# Autodesk Inventor assembly: Humanóide - rev0
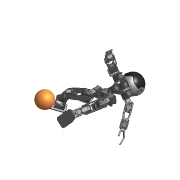
[picture p0: Inventor's stored thumbnail of the model, 180x180]
Saved by Autodesk Inventor 2011 (Build 150239000, 239)
## iProperties
Created: 2010-11-21
Part Number: Humanóide - rev0
Document SubType Name: Assembly
Designer: Milton
Mass: 1911.62 g
Surface Area: 4804 cm^2
Volume: 1270.78 cm^3
Density: 1.50429 g/cm^3
Author: Milton
## Documents named in this file (30)
- C:\Users\Milton\Documents\Futbots\IC - Humanóide\Desenhos\Humanóide - rev0.iam
- C:\Users\Milton\Documents\Futbots\IC - Humanóide\Desenhos\Right foot.ipt
- C:\Users\Milton\Documents\Futbots\IC - Humanóide\Desenhos\Imported Components\RX-28\RX-28.ipt
- C:\Users\Milton\Documents\Futbots\IC - Humanóide\Desenhos\Imported Components\RX-28 Horn\RX-28 Horn.ipt
- C:\Users\Milton\Documents\Futbots\IC - Humanóide\Desenhos\Ankle.ipt
- C:\Users\Milton\Documents\Futbots\IC - Humanóide\Desenhos\Hips.ipt
- C:\Users\Milton\Documents\Futbots\IC - Humanóide\Desenhos\Thigh.ipt
- C:\Users\Milton\Documents\Futbots\IC - Humanóide\Desenhos\Left foot.ipt
- C:\Users\Milton\Documents\Futbots\IC - Humanóide\Desenhos\Knee - Back.ipt
- C:\Users\Milton\Documents\Futbots\IC - Humanóide\Desenhos\Knee - Front.ipt
- C:\Users\Milton\Documents\Futbots\IC - Humanóide\Desenhos\Groin.ipt
- C:\Users\Milton\Documents\Futbots\IC - Humanóide\Desenhos\Pelvis.ipt
- C:\Users\Milton\Documents\Futbots\IC - Humanóide\Desenhos\Waistline.ipt
- C:\Users\Milton\Documents\Futbots\IC - Humanóide\Desenhos\Trunk.ipt
- C:\Users\Milton\Documents\Futbots\IC - Humanóide\Desenhos\Shoulder.ipt
- C:\Users\Milton\Documents\Futbots\IC - Humanóide\Desenhos\Arm.ipt
- C:\Users\Milton\Documents\Futbots\IC - Humanóide\Desenhos\Trapezium.ipt
- C:\Users\Milton\Documents\Futbots\IC - Humanóide\Desenhos\Right Hand.ipt
- C:\Users\Milton\Documents\Futbots\IC - Humanóide\Desenhos\Left Hand.ipt
- C:\Users\Milton\Documents\Futbots\IC - Humanóide\Desenhos\Alça.ipt
- C:\Users\Milton\Documents\Futbots\IC - Humanóide\Desenhos\Neck.ipt
- C:\Users\Milton\Documents\Inventor\Content Center Files\R2011\en-US\ISO 7380\ISO 7380 - M3 x 6.ipt
- C:\Users\Milton\Documents\Futbots\IC - Humanóide\Desenhos\Head.iam
- C:\Users\Milton\Documents\Futbots\IC - Humanóide\Desenhos\Ball.ipt
- C:\Users\Milton\Documents\Futbots\IC - Humanóide\Desenhos\Humanóide - rev0\AIP\Stress Analysis\{6B0C443B-3575-4766-89EC-E2AB749BE7BF}\Brep_0\Humanóide - rev0_INS_{7D960F55-6937-454E-B973-146CFB6E3506}.fins
- C:\Users\Milton\Documents\Futbots\IC - Humanóide\Desenhos\Humanóide - rev0\AIP\Stress Analysis\{6B0C443B-3575-4766-89EC-E2AB749BE7BF}\Brep_0\Humanóide - rev0_sat_{44389967-61AA-4BE1-B7EC-D3EA2D2FE9C6}.fsat
- C:\Users\Milton\Documents\Futbots\IC - Humanóide\Desenhos\Humanóide - rev0\AIP\Stress Analysis\{6B0C443B-3575-4766-89EC-E2AB749BE7BF}\Brep_0\Humanóide - rev0_tes_{B0B6FCF0-E664-439E-BE88-AB80D02FF4B7}.ftes
- C:\Users\Milton\Documents\Futbots\IC - Humanóide\Desenhos\Humanóide - rev0\AIP\Stress Analysis\{6B0C443B-3575-4766-89EC-E2AB749BE7BF}\Brep_0\Humanóide - rev0_wiz_{24C38105-2EA3-4ABB-8DFC-E581D1C3461D}.fwiz
- C:\Users\Milton\Documents\Futbots\IC - Humanóide\Desenhos\Humanóide - rev0\AIP\Stress Analysis\{6B0C443B-3575-4766-89EC-E2AB749BE7BF}\Simulation_0\Humanóide - rev0_msh_{642BD46C-0DBD-4A00-9AC0-F0BB7B45041F}.fmsh
- C:\Users\Milton\Documents\Futbots\IC - Humanóide\Desenhos\Humanóide - rev0\AIP\Stress Analysis\{6B0C443B-3575-4766-89EC-E2AB749BE7BF}\Simulation_0\Humanóide - rev0_res_{B27E6E0C-00E3-4C61-99AA-CF472A861E25}.fres
## Components (147 placed, 23 different names)
1. RX-28:1 — Mate:58, Mate:59, Mate:60, Mate:67, Mate:68, Mate:73
2. RX-28:2 — Mate:55, Mate:56, Mate:57, Mate:69, Mate:70, Mate:76
3. RX-28:3 — Mate:80, Mate:81, Mate:82, Mate:83, Mate:84, Mate:85, Mate:86, Mate:87, Flush:7, Mate:128, Mate:211
4. RX-28:4 — Mate:88, Mate:89, Mate:90, Mate:97, Mate:98, Flush:9, Mate:129, Mate:130, Flush:13, Insert:22, Insert:23
5. RX-28:5 — Mate:91, Mate:92, Mate:93, Mate:95, Mate:96, Mate:131, Mate:200, Mate:201, Insert:37, Insert:38, Insert:62
6. RX-28:6 — Flush:7, Mate:128, Flush:9, Mate:132, Mate:133, Mate:196, Mate:197
7. RX-28 Horn:1 — Mate:4, Mate:5, Mate:159, Mate:160, Mate:161
8. RX-28 Horn:2 — Mate:6, Mate:7, Mate:180, Mate:181, Mate:182, Mate:194, Mate:195
9. RX-28 Horn:3 — Mate:8, Mate:10, Mate:12, Mate:14, Flush:3, Flush:4, Mate:31
10. RX-28 Horn:4 — Mate:16, Mate:19, Mate:20, Flush:5, Flush:6, Mate:34
11. RX-28 Horn:5 — Mate:15, Mate:17, Mate:18, Mate:21, Mate:177, Mate:178, Mate:179, Mate:191, Mate:192, Mate:193, Insert:9, Insert:10, Insert:48, Insert:49, Insert:85, Insert:86
12. RX-28 Horn:6 — Mate:32, Flush:5, Flush:6, Mate:127
13. RX-28 Horn:7 — Mate:99, Mate:100, Flush:10, Mate:168, Mate:169, Mate:170, Mate:171, Mate:172
14. RX-28 Horn:8 — Mate:27, Mate:28, Mate:175, Mate:184, Mate:185, Mate:189, Mate:190
15. RX-28 Horn:9 — Mate:101, Mate:102, Mate:144, Mate:145, Mate:147, Mate:148, Mate:164, Mate:165
16. RX-28 Horn:10 — Mate:9, Mate:11, Mate:13, Mate:173, Mate:174, Mate:183, Mate:186, Mate:187, Mate:188, Insert:11, Insert:12, Insert:46, Insert:47, Insert:77, Insert:79, Insert:83, Insert:84
17. RX-28 Horn:11 — Flush:10, Mate:141, Mate:153, Mate:154, Mate:155, Mate:166, Mate:167, Insert:42, Insert:43, Insert:91, Insert:92
18. RX-28 Horn:16 — Mate:61, Mate:62, Mate:63, Mate:64, Mate:65, Mate:66, Mate:72, Mate:74, Mate:75, Mate:77, Mate:78, Mate:79, Mate:212
19. RX-28 Horn:17 — Mate:29, Flush:3, Flush:4, Mate:126
20. RX-28 Horn:19 — Mate:149, Mate:150, Mate:156, Mate:157, Mate:208, Insert:87, Insert:88, Insert:89, Insert:90
21. RX-28 Horn:21 — Mate:22, Mate:25, Mate:26, Mate:162, Mate:163
22. RX-28 Horn:22 — Mate:198, Mate:199, Mate:213
23. Ankle:1 — Mate:4, Mate:5, Mate:6, Mate:7
24. Ankle:2 — Mate:25, Mate:26, Mate:27, Mate:28
25. Hips:1 — Mate:32, Mate:34, Mate:69, Mate:70, Mate:127
26. Hips:2 — Mate:29, Mate:31, Mate:67, Mate:68, Mate:126
27. Thigh:1 — Mate:8, Mate:9, Mate:10, Mate:11
28. Thigh:2 — Mate:12, Mate:13, Mate:14
29. Thigh:3 — Mate:15, Mate:16, Mate:17
30. Thigh:4 — Mate:18, Mate:19, Mate:20, Mate:21
31. Waistline:1 — Mate:78, Mate:79, Mate:80, Mate:81
32. Right foot:1 — Mate:159, Mate:160, Mate:161, Insert:16, Insert:17, Insert:68, Insert:69, Mate:210
33. Left foot:1 — Mate:22, Mate:162, Mate:163, Mate:202, Mate:203, Insert:15, Insert:70, Insert:71, Insert:72, Mate:209
34. Knee - Back:1 — Mate:186, Mate:187, Mate:188, Mate:189, Mate:190, Insert:18, Insert:19
35. Knee - Front:1 — Mate:173, Mate:174, Mate:175, Mate:183, Mate:184, Mate:185, Insert:75, Insert:76
36. Knee - Front:2 — Mate:177, Mate:178, Mate:179, Mate:180, Mate:181, Mate:182, Insert:73, Insert:74
37. Groin:1 — Mate:55, Mate:56, Mate:57, Mate:64, Mate:65, Mate:66, Insert:32, Insert:36, Insert:52, Insert:53
38. Groin:2 — Mate:58, Mate:59, Mate:60, Mate:61, Mate:62, Mate:63, Insert:44, Insert:45, Insert:50, Insert:51
39. Pelvis:1 — Mate:75, Mate:76, Mate:77, Insert:30, Insert:31, Insert:34, Insert:35
40. Pelvis:2 — Mate:72, Mate:73, Mate:74, Insert:13, Insert:14, Insert:33, Mate:204, Mate:205
41. Trunk:1 — Mate:82, Mate:83, Mate:84, Mate:88, Mate:89, Mate:90, Insert:28, Insert:29, Insert:54, Insert:55
42. Trunk:2 — Mate:85, Mate:86, Mate:87, Mate:91, Mate:92, Mate:93, Insert:24, Insert:25, Insert:26, Insert:27
43. Shoulder:1 — Mate:97, Mate:98, Mate:101, Mate:102
44. Shoulder:2 — Mate:95, Mate:96, Mate:99, Mate:100
45. Trapezium:1 — Mate:129, Mate:130, Insert:56, Insert:57, Insert:58, Insert:63
46. Trapezium:2 — Mate:131, Mate:132, Mate:133, Insert:59, Insert:60
47. Right Hand:1 — Mate:153, Mate:154, Mate:155
48. Arm:3 — Mate:170, Mate:171, Mate:172, Insert:39, Insert:40, Mate:206, Mate:207, Insert:41
49. Arm:4 — Mate:147, Mate:148, Mate:165, Insert:5, Insert:6, Insert:7, Insert:8
50. Arm:6 — Mate:141, Mate:166, Mate:167, Mate:168, Mate:169, Insert:64, Insert:65, Insert:66, Insert:67
51. Arm:7 — Mate:144, Mate:145, Mate:149, Mate:150, Mate:164, Insert:1, Insert:2, Insert:3, Insert:4
52. Left Hand:1 — Mate:156, Mate:157, Mate:208
53. Knee - Back:2 — Mate:191, Mate:192, Mate:193, Mate:194, Mate:195, Insert:20, Insert:21
54. Alça:1 — Flush:13, Mate:200, Mate:201
55. Neck:1 — Mate:196, Mate:197, Mate:198, Mate:199, Flush:14
56. Head:1 [sub-assembly] — Mate:213, Flush:14
57. Ball:1
58. ISO 7380 M3 x 6:1 — Insert:1
59. ISO 7380 M3 x 6:2 — Insert:2
60. ISO 7380 M3 x 6:3 — Insert:3
61. ISO 7380 M3 x 6:4 — Insert:4
62. ISO 7380 M3 x 6:5 — Insert:5
63. ISO 7380 M3 x 6:6 — Insert:6
64. ISO 7380 M3 x 6:7 — Insert:7
65. ISO 7380 M3 x 6:8 — Insert:8
66. ISO 7380 M3 x 6:9 — Insert:9
67. ISO 7380 M3 x 6:10 — Insert:10
68. ISO 7380 M3 x 6:11 — Insert:11
69. ISO 7380 M3 x 6:12 — Insert:12
70. ISO 7380 M3 x 6:13 — Insert:13
71. ISO 7380 M3 x 6:14 — Insert:14
72. ISO 7380 M3 x 6:15 — Mate:202, Mate:203
73. ISO 7380 M3 x 6:16 — Insert:15
74. ISO 7380 M3 x 6:17 — Insert:16
75. ISO 7380 M3 x 6:18 — Insert:17
76. ISO 7380 M3 x 6:19 — Insert:18
77. ISO 7380 M3 x 6:20 — Insert:19
78. ISO 7380 M3 x 6:21 — Insert:20
79. ISO 7380 M3 x 6:22 — Insert:21
80. ISO 7380 M3 x 6:23 — Insert:22
81. ISO 7380 M3 x 6:24 — Insert:23
82. ISO 7380 M3 x 6:25 — Insert:24
83. ISO 7380 M3 x 6:26 — Insert:25
84. ISO 7380 M3 x 6:27 — Insert:26
85. ISO 7380 M3 x 6:28 — Insert:27
86. ISO 7380 M3 x 6:29 — Insert:28
87. ISO 7380 M3 x 6:30 — Insert:29
88. ISO 7380 M3 x 6:31 — Insert:30
89. ISO 7380 M3 x 6:32 — Insert:31
90. ISO 7380 M3 x 6:33 — Insert:32
91. ISO 7380 M3 x 6:34 — Insert:33
92. ISO 7380 M3 x 6:35 — Mate:204, Mate:205
93. ISO 7380 M3 x 6:36 — Insert:34
94. ISO 7380 M3 x 6:37 — Insert:35
95. ISO 7380 M3 x 6:38 — Insert:36
96. ISO 7380 M3 x 6:39 — Insert:37
97. ISO 7380 M3 x 6:40 — Insert:38
98. ISO 7380 M3 x 6:41 — Insert:39
99. ISO 7380 M3 x 6:42 — Insert:40
100. ISO 7380 M3 x 6:43 — Mate:206, Mate:207
101. ISO 7380 M3 x 6:44 — Insert:41
102. ISO 7380 M3 x 6:45 — Insert:42
103. ISO 7380 M3 x 6:46 — Insert:43
104. ISO 7380 M3 x 6:47 — Insert:44
105. ISO 7380 M3 x 6:48 — Insert:45
106. ISO 7380 M3 x 6:49 — Insert:46
107. ISO 7380 M3 x 6:50 — Insert:47
108. ISO 7380 M3 x 6:51 — Insert:48
109. ISO 7380 M3 x 6:52 — Insert:49
110. ISO 7380 M3 x 6:53 — Insert:50
111. ISO 7380 M3 x 6:54 — Insert:51
112. ISO 7380 M3 x 6:55 — Insert:52
113. ISO 7380 M3 x 6:56 — Insert:53
114. ISO 7380 M3 x 6:57 — Insert:54
115. ISO 7380 M3 x 6:58 — Insert:55
116. ISO 7380 M3 x 6:59 — Insert:56
117. ISO 7380 M3 x 6:60 — Insert:57
118. ISO 7380 M3 x 6:61 — Insert:58
119. ISO 7380 M3 x 6:62 — Insert:59
120. ISO 7380 M3 x 6:63 — Insert:60
121. ISO 7380 M3 x 6:65 — Insert:62
122. ISO 7380 M3 x 6:66 — Insert:63
123. ISO 7380 M3 x 6:67 — Insert:64
124. ISO 7380 M3 x 6:68 — Insert:65
125. ISO 7380 M3 x 6:69 — Insert:66
126. ISO 7380 M3 x 6:70 — Insert:67
127. ISO 7380 M3 x 6:71 — Insert:68
128. ISO 7380 M3 x 6:72 — Insert:69
129. ISO 7380 M3 x 6:73 — Insert:70
130. ISO 7380 M3 x 6:74 — Insert:71
131. ISO 7380 M3 x 6:75 — Insert:72
132. ISO 7380 M3 x 6:76 — Insert:73
133. ISO 7380 M3 x 6:77 — Insert:74
134. ISO 7380 M3 x 6:78 — Insert:75
135. ISO 7380 M3 x 6:79 — Insert:76
136. ISO 7380 M3 x 6:80 — Insert:77
137. ISO 7380 M3 x 6:82 — Insert:79
138. ISO 7380 M3 x 6:86 — Insert:83
139. ISO 7380 M3 x 6:87 — Insert:84
140. ISO 7380 M3 x 6:88 — Insert:85
141. ISO 7380 M3 x 6:89 — Insert:86
142. ISO 7380 M3 x 6:90 — Insert:87
143. ISO 7380 M3 x 6:91 — Insert:88
144. ISO 7380 M3 x 6:92 — Insert:89
145. ISO 7380 M3 x 6:93 — Insert:90
146. ISO 7380 M3 x 6:94 — Insert:91
147. ISO 7380 M3 x 6:95 — Insert:92
## Relationships (243: Mate 147, Insert 87, Flush 9)
- Mate:4: RX-28 Horn:1 ↔ Ankle:1
- Mate:5: RX-28 Horn:1 ↔ Ankle:1
- Mate:6: RX-28 Horn:2 ↔ Ankle:1
- Mate:7: RX-28 Horn:2 ↔ Ankle:1
- Mate:8: RX-28 Horn:3 ↔ Thigh:1
- Mate:9: RX-28 Horn:10 ↔ Thigh:1
- Mate:10: RX-28 Horn:3 ↔ Thigh:1
- Mate:11: RX-28 Horn:10 ↔ Thigh:1
- Mate:12: RX-28 Horn:3 ↔ Thigh:2
- Mate:13: RX-28 Horn:10 ↔ Thigh:2
- Mate:14: RX-28 Horn:3 ↔ Thigh:2
- Mate:15: RX-28 Horn:5 ↔ Thigh:3
- Mate:16: RX-28 Horn:4 ↔ Thigh:3
- Mate:17: RX-28 Horn:5 ↔ Thigh:3
- Mate:18: RX-28 Horn:5 ↔ Thigh:4
- Mate:19: RX-28 Horn:4 ↔ Thigh:4
- Mate:20: RX-28 Horn:4 ↔ Thigh:4
- Mate:21: RX-28 Horn:5 ↔ Thigh:4
- Mate:22: RX-28 Horn:21 ↔ Left foot:1
- Mate:25: RX-28 Horn:21 ↔ Ankle:2
- Mate:26: RX-28 Horn:21 ↔ Ankle:2
- Mate:27: RX-28 Horn:8 ↔ Ankle:2
- Mate:28: RX-28 Horn:8 ↔ Ankle:2
- Mate:29: RX-28 Horn:17 ↔ Hips:2
- Flush:3: RX-28 Horn:3 ↔ RX-28 Horn:17
- Flush:4: RX-28 Horn:3 ↔ RX-28 Horn:17
- Mate:31 (3 mm): RX-28 Horn:3 ↔ Hips:2
- Mate:32: RX-28 Horn:6 ↔ Hips:1
- Flush:5: RX-28 Horn:4 ↔ RX-28 Horn:6
- Flush:6: RX-28 Horn:4 ↔ RX-28 Horn:6
- Mate:34 (3 mm): RX-28 Horn:4 ↔ Hips:1
- Mate:55: RX-28:2 ↔ Groin:1
- Mate:56: RX-28:2 ↔ Groin:1
- Mate:57: RX-28:2 ↔ Groin:1
- Mate:58: RX-28:1 ↔ Groin:2
- Mate:59: RX-28:1 ↔ Groin:2
- Mate:60: RX-28:1 ↔ Groin:2
- Mate:61: RX-28 Horn:16 ↔ Groin:2
- Mate:62: RX-28 Horn:16 ↔ Groin:2
- Mate:63: RX-28 Horn:16 ↔ Groin:2
- Mate:64: RX-28 Horn:16 ↔ Groin:1
- Mate:65: RX-28 Horn:16 ↔ Groin:1
- Mate:66: RX-28 Horn:16 ↔ Groin:1
- Mate:67: RX-28:1 ↔ Hips:2
- Mate:68: RX-28:1 ↔ Hips:2
- Mate:69: RX-28:2 ↔ Hips:1
- Mate:70: RX-28:2 ↔ Hips:1
- Mate:72: RX-28 Horn:16 ↔ Pelvis:2
- Mate:73: RX-28:1 ↔ Pelvis:2
- Mate:74: RX-28 Horn:16 ↔ Pelvis:2
- Mate:75: RX-28 Horn:16 ↔ Pelvis:1
- Mate:76: RX-28:2 ↔ Pelvis:1
- Mate:77: RX-28 Horn:16 ↔ Pelvis:1
- Mate:78: RX-28 Horn:16 ↔ Waistline:1
- Mate:79: RX-28 Horn:16 ↔ Waistline:1
- Mate:80: RX-28:3 ↔ Waistline:1
- Mate:81: RX-28:3 ↔ Waistline:1
- Mate:82: RX-28:3 ↔ Trunk:1
- Mate:83: RX-28:3 ↔ Trunk:1
- Mate:84: RX-28:3 ↔ Trunk:1
- Mate:85: RX-28:3 ↔ Trunk:2
- Mate:86: RX-28:3 ↔ Trunk:2
- Mate:87: RX-28:3 ↔ Trunk:2
- Mate:88: RX-28:4 ↔ Trunk:1
- Mate:89: RX-28:4 ↔ Trunk:1
- Mate:90: RX-28:4 ↔ Trunk:1
- Mate:91: RX-28:5 ↔ Trunk:2
- Mate:92: RX-28:5 ↔ Trunk:2
- Mate:93: RX-28:5 ↔ Trunk:2
- Mate:95: RX-28:5 ↔ Shoulder:2
- Mate:96: RX-28:5 ↔ Shoulder:2
- Mate:97: RX-28:4 ↔ Shoulder:1
- Mate:98: RX-28:4 ↔ Shoulder:1
- Mate:99: RX-28 Horn:7 ↔ Shoulder:2
- Mate:100: RX-28 Horn:7 ↔ Shoulder:2
- Mate:101: RX-28 Horn:9 ↔ Shoulder:1
- Mate:102: RX-28 Horn:9 ↔ Shoulder:1
- Mate:126: RX-28 Horn:17 ↔ Hips:2
- Mate:127: RX-28 Horn:6 ↔ Hips:1
- Flush:7: RX-28:3 ↔ RX-28:6
- Mate:128: RX-28:3 ↔ RX-28:6
- Flush:9: RX-28:4 ↔ RX-28:6
- Mate:129: RX-28:4 ↔ Trapezium:1
- Mate:130: RX-28:4 ↔ Trapezium:1
- Mate:131: RX-28:5 ↔ Trapezium:2
- Mate:132: RX-28:6 ↔ Trapezium:2
- Mate:133: RX-28:6 ↔ Trapezium:2
- Flush:10: RX-28 Horn:7 ↔ RX-28 Horn:11
- Mate:141: RX-28 Horn:11 ↔ Arm:6
- Mate:144: RX-28 Horn:9 ↔ Arm:7
- Mate:145: RX-28 Horn:9 ↔ Arm:7
- Mate:147: RX-28 Horn:9 ↔ Arm:4
- Mate:148: RX-28 Horn:9 ↔ Arm:4
- Mate:149: RX-28 Horn:19 ↔ Arm:7
- Mate:150: RX-28 Horn:19 ↔ Arm:7
- Mate:153: RX-28 Horn:11 ↔ Right Hand:1
- Mate:154: RX-28 Horn:11 ↔ Right Hand:1
- Mate:155: RX-28 Horn:11 ↔ Right Hand:1
- Mate:156: RX-28 Horn:19 ↔ Left Hand:1
- Mate:157: RX-28 Horn:19 ↔ Left Hand:1
- Mate:159: RX-28 Horn:1 ↔ Right foot:1
- Mate:160: RX-28 Horn:1 ↔ Right foot:1
- Mate:161: RX-28 Horn:1 ↔ Right foot:1
- Mate:162: RX-28 Horn:21 ↔ Left foot:1
- Mate:163: RX-28 Horn:21 ↔ Left foot:1
- Mate:164: RX-28 Horn:9 ↔ Arm:7
- Mate:165: RX-28 Horn:9 ↔ Arm:4
- Mate:166: RX-28 Horn:11 ↔ Arm:6
- Mate:167: RX-28 Horn:11 ↔ Arm:6
- Mate:168: RX-28 Horn:7 ↔ Arm:6
- Mate:169: RX-28 Horn:7 ↔ Arm:6
- Mate:170: RX-28 Horn:7 ↔ Arm:3
- Mate:171: RX-28 Horn:7 ↔ Arm:3
- Mate:172: RX-28 Horn:7 ↔ Arm:3
- Mate:173: RX-28 Horn:10 ↔ Knee - Front:1
- Mate:174: RX-28 Horn:10 ↔ Knee - Front:1
- Mate:175: RX-28 Horn:8 ↔ Knee - Front:1
- Mate:177: RX-28 Horn:5 ↔ Knee - Front:2
- Mate:178: RX-28 Horn:5 ↔ Knee - Front:2
- Mate:179: RX-28 Horn:5 ↔ Knee - Front:2
- Mate:180: RX-28 Horn:2 ↔ Knee - Front:2
- Mate:181: RX-28 Horn:2 ↔ Knee - Front:2
- Mate:182: RX-28 Horn:2 ↔ Knee - Front:2
- Mate:183: RX-28 Horn:10 ↔ Knee - Front:1
- Mate:184: RX-28 Horn:8 ↔ Knee - Front:1
- Mate:185: RX-28 Horn:8 ↔ Knee - Front:1
- Mate:186: RX-28 Horn:10 ↔ Knee - Back:1
- Mate:187: RX-28 Horn:10 ↔ Knee - Back:1
- Mate:188: RX-28 Horn:10 ↔ Knee - Back:1
- Mate:189: RX-28 Horn:8 ↔ Knee - Back:1
- Mate:190: RX-28 Horn:8 ↔ Knee - Back:1
- Mate:191: RX-28 Horn:5 ↔ Knee - Back:2
- Mate:192: RX-28 Horn:5 ↔ Knee - Back:2
- Mate:193: RX-28 Horn:5 ↔ Knee - Back:2
- Mate:194: RX-28 Horn:2 ↔ Knee - Back:2
- Mate:195: RX-28 Horn:2 ↔ Knee - Back:2
- Flush:13: RX-28:4 ↔ Alça:1
- Mate:196: RX-28:6 ↔ Neck:1
- Mate:197: RX-28:6 ↔ Neck:1
- Mate:198: RX-28 Horn:22 ↔ Neck:1
- Mate:199: RX-28 Horn:22 ↔ Neck:1
- Mate:200: RX-28:5 ↔ Alça:1
- Mate:201: RX-28:5 ↔ Alça:1
- Mate:203: Left foot:1 ↔ ISO 7380 M3 x 6:15
- Mate:205: Pelvis:2 ↔ ISO 7380 M3 x 6:35
- Mate:207: Arm:3 ↔ ISO 7380 M3 x 6:43
- Mate:208: RX-28 Horn:19 ↔ Left Hand:1
- Mate:209: Left foot:1
- Mate:210: Right foot:1
- Mate:211: RX-28:3
- Mate:212 (-15 mm): RX-28 Horn:16
- Mate:213: RX-28 Horn:22 ↔ Head:1
- Flush:14 (-35.5 mm): Neck:1 ↔ Head:1
- Insert:1: Arm:7 ↔ ISO 7380 M3 x 6:1
- Insert:2: Arm:7 ↔ ISO 7380 M3 x 6:2
- Insert:3: Arm:7 ↔ ISO 7380 M3 x 6:3
- Insert:4: Arm:7 ↔ ISO 7380 M3 x 6:4
- Insert:5: Arm:4 ↔ ISO 7380 M3 x 6:5
- Insert:6: Arm:4 ↔ ISO 7380 M3 x 6:6
- Insert:7: Arm:4 ↔ ISO 7380 M3 x 6:7
- Insert:8: Arm:4 ↔ ISO 7380 M3 x 6:8
- Insert:9: RX-28 Horn:5 ↔ ISO 7380 M3 x 6:9
- Insert:10: RX-28 Horn:5 ↔ ISO 7380 M3 x 6:10
- Insert:11: RX-28 Horn:10 ↔ ISO 7380 M3 x 6:11
- Insert:12: RX-28 Horn:10 ↔ ISO 7380 M3 x 6:12
- Insert:13: Pelvis:2 ↔ ISO 7380 M3 x 6:13
- Insert:14: Pelvis:2 ↔ ISO 7380 M3 x 6:14
- Mate:202: Left foot:1 ↔ ISO 7380 M3 x 6:15
- Insert:15: Left foot:1 ↔ ISO 7380 M3 x 6:16
- Insert:16: Right foot:1 ↔ ISO 7380 M3 x 6:17
- Insert:17: Right foot:1 ↔ ISO 7380 M3 x 6:18
- Insert:18: Knee - Back:1 ↔ ISO 7380 M3 x 6:19
- Insert:19: Knee - Back:1 ↔ ISO 7380 M3 x 6:20
- Insert:20: Knee - Back:2 ↔ ISO 7380 M3 x 6:21
- Insert:21: Knee - Back:2 ↔ ISO 7380 M3 x 6:22
- Insert:22: RX-28:4 ↔ ISO 7380 M3 x 6:23
- Insert:23: RX-28:4 ↔ ISO 7380 M3 x 6:24
- Insert:24: Trunk:2 ↔ ISO 7380 M3 x 6:25
- Insert:25: Trunk:2 ↔ ISO 7380 M3 x 6:26
- Insert:26: Trunk:2 ↔ ISO 7380 M3 x 6:27
- Insert:27: Trunk:2 ↔ ISO 7380 M3 x 6:28
- Insert:28: Trunk:1 ↔ ISO 7380 M3 x 6:29
- Insert:29: Trunk:1 ↔ ISO 7380 M3 x 6:30
- Insert:30: Pelvis:1 ↔ ISO 7380 M3 x 6:31
- Insert:31: Pelvis:1 ↔ ISO 7380 M3 x 6:32
- Insert:32: Groin:1 ↔ ISO 7380 M3 x 6:33
- Insert:33: Pelvis:2 ↔ ISO 7380 M3 x 6:34
- Mate:204: Pelvis:2 ↔ ISO 7380 M3 x 6:35
- Insert:34: Pelvis:1 ↔ ISO 7380 M3 x 6:36
- Insert:35: Pelvis:1 ↔ ISO 7380 M3 x 6:37
- Insert:36: Groin:1 ↔ ISO 7380 M3 x 6:38
- Insert:37: RX-28:5 ↔ ISO 7380 M3 x 6:39
- Insert:38: RX-28:5 ↔ ISO 7380 M3 x 6:40
- Insert:39: Arm:3 ↔ ISO 7380 M3 x 6:41
- Insert:40: Arm:3 ↔ ISO 7380 M3 x 6:42
- Mate:206: Arm:3 ↔ ISO 7380 M3 x 6:43
- Insert:41: Arm:3 ↔ ISO 7380 M3 x 6:44
- Insert:42: RX-28 Horn:11 ↔ ISO 7380 M3 x 6:45
- Insert:43: RX-28 Horn:11 ↔ ISO 7380 M3 x 6:46
- Insert:44: Groin:2 ↔ ISO 7380 M3 x 6:47
- Insert:45: Groin:2 ↔ ISO 7380 M3 x 6:48
- Insert:46: RX-28 Horn:10 ↔ ISO 7380 M3 x 6:49
- Insert:47: RX-28 Horn:10 ↔ ISO 7380 M3 x 6:50
- Insert:48: RX-28 Horn:5 ↔ ISO 7380 M3 x 6:51
- Insert:49: RX-28 Horn:5 ↔ ISO 7380 M3 x 6:52
- Insert:50: Groin:2 ↔ ISO 7380 M3 x 6:53
- Insert:51: Groin:2 ↔ ISO 7380 M3 x 6:54
- Insert:52: Groin:1 ↔ ISO 7380 M3 x 6:55
- Insert:53: Groin:1 ↔ ISO 7380 M3 x 6:56
- Insert:54: Trunk:1 ↔ ISO 7380 M3 x 6:57
- Insert:55: Trunk:1 ↔ ISO 7380 M3 x 6:58
- Insert:56: Trapezium:1 ↔ ISO 7380 M3 x 6:59
- Insert:57: Trapezium:1 ↔ ISO 7380 M3 x 6:60
- Insert:58: Trapezium:1 ↔ ISO 7380 M3 x 6:61
- Insert:59: Trapezium:2 ↔ ISO 7380 M3 x 6:62
- Insert:60: Trapezium:2 ↔ ISO 7380 M3 x 6:63
- Insert:62: RX-28:5 ↔ ISO 7380 M3 x 6:65
- Insert:63: Trapezium:1 ↔ ISO 7380 M3 x 6:66
- Insert:64: Arm:6 ↔ ISO 7380 M3 x 6:67
- Insert:65: Arm:6 ↔ ISO 7380 M3 x 6:68
- Insert:66: Arm:6 ↔ ISO 7380 M3 x 6:69
- Insert:67: Arm:6 ↔ ISO 7380 M3 x 6:70
- Insert:68: Right foot:1 ↔ ISO 7380 M3 x 6:71
- Insert:69: Right foot:1 ↔ ISO 7380 M3 x 6:72
- Insert:70: Left foot:1 ↔ ISO 7380 M3 x 6:73
- Insert:71: Left foot:1 ↔ ISO 7380 M3 x 6:74
- Insert:72: Left foot:1 ↔ ISO 7380 M3 x 6:75
- Insert:73: Knee - Front:2 ↔ ISO 7380 M3 x 6:76
- Insert:74: Knee - Front:2 ↔ ISO 7380 M3 x 6:77
- Insert:75: Knee - Front:1 ↔ ISO 7380 M3 x 6:78
- Insert:76: Knee - Front:1 ↔ ISO 7380 M3 x 6:79
- Insert:77: RX-28 Horn:10 ↔ ISO 7380 M3 x 6:80
- Insert:79: RX-28 Horn:10 ↔ ISO 7380 M3 x 6:82
- Insert:83: RX-28 Horn:10 ↔ ISO 7380 M3 x 6:86
- Insert:84: RX-28 Horn:10 ↔ ISO 7380 M3 x 6:87
- Insert:85: RX-28 Horn:5 ↔ ISO 7380 M3 x 6:88
- Insert:86: RX-28 Horn:5 ↔ ISO 7380 M3 x 6:89
- Insert:87: RX-28 Horn:19 ↔ ISO 7380 M3 x 6:90
- Insert:88: RX-28 Horn:19 ↔ ISO 7380 M3 x 6:91
- Insert:89: RX-28 Horn:19 ↔ ISO 7380 M3 x 6:92
- Insert:90: RX-28 Horn:19 ↔ ISO 7380 M3 x 6:93
- Insert:91: RX-28 Horn:11 ↔ ISO 7380 M3 x 6:94
- Insert:92: RX-28 Horn:11 ↔ ISO 7380 M3 x 6:95
